# Autodesk Inventor assembly: zDrive
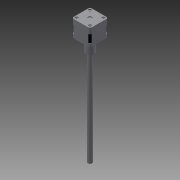
[picture p0: Inventor's stored thumbnail of the model, 180x180]
Saved by Autodesk Inventor 2013 (Build 170138000, 138)
## iProperties
Created: 2015-01-14
Part Number: zDrive
Document SubType Name: Assembly
Designer: dzban
Author: dzban
## Documents named in this file (4)
- D:\PIRX\Artisan\OPENSOURCE\ZCar\zDrive.iam
- D:\PIRX\Artisan\OPENSOURCE\StockComponents\flexibleShaftCoupling.ipt
- D:\PIRX\Artisan\OPENSOURCE\StockComponents\NEMA17Stepper.ipt
- D:\PIRX\Artisan\OPENSOURCE\ZCar\trapeziodialScrew10x2.ipt
## Components (3 placed, 3 different names)
1. flexibleShaftCoupling:1 — Insert:1, Insert:2
2. NEMA17Stepper:1 — Insert:1
3. trapeziodialScrew10x2:1 — Insert:2
## Relationships (2: Insert 2)
- Insert:1 (2 mm): flexibleShaftCoupling:1 ↔ NEMA17Stepper:1
- Insert:2 (-10 mm): flexibleShaftCoupling:1 ↔ trapeziodialScrew10x2:1
